# Autodesk Inventor assembly: SprocketAdapter_assembly
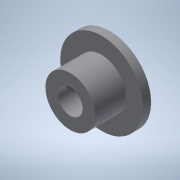
[picture p0: Inventor's stored thumbnail of the model, 180x180]
Saved by Autodesk Inventor 2021 (Build 250183000, 183)
## iProperties
Created: 2020-09-20
Part Number: SprocketAdapter_assembly
Document SubType Name: Assembly
Designer: PhotonUser
Author: PhotonUser
Quantity: 1
## Documents named in this file (3)
- D:\PhotonUser\Downloads\Assembly Files-20200920T011428Z-001\Assembly Files\SprocketAdapter_assembly.iam
- D:\PhotonUser\Downloads\Assembly Files-20200920T011428Z-001\Assembly Files\WoodruffKey.ipt
- D:\PhotonUser\Downloads\Assembly Files-20200920T011428Z-001\Assembly Files\SprocketAdapter.ipt
## Components (2 placed, 2 different names)
1. WoodruffKey:1 — Mate:1, Tangent:1, Mate:2
2. SprocketAdapter:1 — Mate:1, Tangent:1, Mate:2
## Relationships (3: Mate 2, Tangent 1)
- Mate:1: WoodruffKey:1 ↔ SprocketAdapter:1
- Tangent:1: WoodruffKey:1 ↔ SprocketAdapter:1
- Mate:2: WoodruffKey:1 ↔ SprocketAdapter:1
